# Autodesk Inventor assembly: Section 2
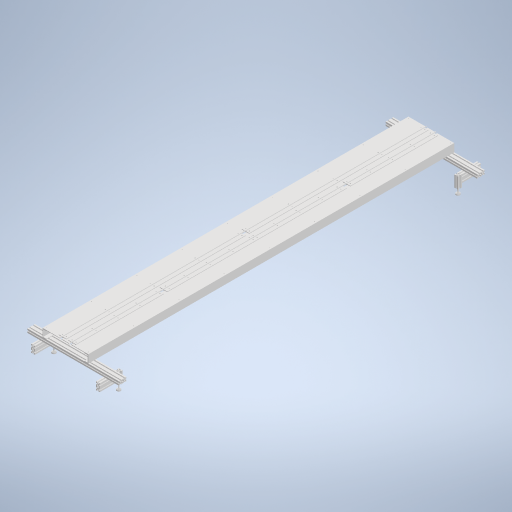
[picture p0: Inventor's stored thumbnail of the model, 512x512]
Saved by Autodesk Inventor 2023 (Build 270158030, 158C)
## iProperties
Created: 2022-06-30
Part Number: Section 2
Document SubType Name: Assembly
Designer: jeremyy
Author: jeremyy
## Documents named in this file (11)
- \\andrew.ad.cmu.edu\users\users1\jeremyy\Documents\Inventor\CMU Bridge\New folder\Section 2.iam
- \\andrew.ad.cmu.edu\users\users1\jeremyy\Documents\Inventor\CMU Bridge\New folder\VertX3in.ipt
- \\andrew.ad.cmu.edu\users\users1\jeremyy\Documents\Inventor\CMU Bridge\New folder\LongXX5.ipt
- \\andrew.ad.cmu.edu\users\users1\jeremyy\Documents\Inventor\CMU Bridge\New folder\LatXX24in.ipt
- \\andrew.ad.cmu.edu\users\users1\jeremyy\Documents\Inventor\CMU Bridge\New folder\LongC96.ipt
- \\andrew.ad.cmu.edu\users\users1\jeremyy\Documents\Inventor\CMU Bridge\New folder\Plate1ftx8ft.ipt
- \\andrew.ad.cmu.edu\users\users1\jeremyy\Documents\Inventor\CMU Bridge\New folder\Foot.ipt
- \\andrew.ad.cmu.edu\users\users1\jeremyy\Documents\Inventor\CMU Bridge\New folder\PlateRailClamp48in.iam
- \\andrew.ad.cmu.edu\users\users1\jeremyy\Documents\Inventor\CMU Bridge\New folder\PlateRail24in.iam
- \\andrew.ad.cmu.edu\users\users1\jeremyy\Documents\Inventor\CMU Bridge\New folder\RailClamp.ipt
- \\andrew.ad.cmu.edu\users\users1\jeremyy\Documents\Inventor\CMU Bridge\New folder\PlateRail23_5.iam
## Components (24 placed, 10 different names)
1. LatXX24in:1 — Flush:1, Flush:2, Mate:1, Flush:3, Mate:2, Flush:4, Mate:4, Flush:7, Flush:8, Mate:5, Flush:26
2. LongXX5:1 — Flush:1, Flush:2, Mate:1, Mate:8, Flush:15, Flush:16
3. LongXX5:2 — Flush:3, Mate:2, Flush:4, Flush:5, Flush:6, Mate:3
4. VertX3in:1 — Flush:5, Flush:6, Mate:3, Mate:13, Tangent:1
5. LongC96:1 — Mate:4, Flush:7, Flush:10, Mate:6, Flush:11
6. LongC96:2 — Flush:8, Mate:5, Flush:12, Mate:7, Flush:13, Flush:25, Flush:26
7. Plate1ftx8ft:1 — Flush:10, Mate:6, Flush:11, Flush:12, Mate:17, Flush:27, Flush:28, Mate:18, Mate:20, Flush:30, Flush:31, Mate:21, Flush:32, Flush:33, Mate:25, Mate:27
8. LatXX24in:2 — Mate:7, Flush:13, Flush:17, Flush:18, Mate:9, Mate:10, Flush:19, Flush:20, Flush:25
9. VertX3in:2 — Mate:8, Flush:15, Flush:16, Mate:14, Tangent:2
10. LongXX5:3 — Flush:17, Flush:18, Mate:9, Flush:23, Mate:12, Flush:24
11. LongXX5:4 — Mate:10, Flush:19, Flush:20, Flush:21, Mate:11, Flush:22
12. VertX3in:3 — Flush:21, Mate:11, Flush:22, Mate:16, Tangent:4
13. VertX3in:4 — Flush:23, Mate:12, Flush:24, Mate:15, Tangent:3
14. Foot:1 — Mate:13, Tangent:1
15. Foot:2 — Mate:14, Tangent:2
16. Foot:3 — Mate:15, Tangent:3
17. Foot:4 — Mate:16, Tangent:4
18. PlateRailClamp48in:1 [sub-assembly] — Mate:17, Flush:27, Flush:28, Mate:19, Flush:29
19. PlateRailClamp48in:2 [sub-assembly] — Mate:18, Mate:19, Flush:29
20. PlateRail24in:1 [sub-assembly] — Mate:20, Flush:30, Flush:31, Mate:26, Flush:34
21. PlateRail24in:2 [sub-assembly] — Mate:21, Flush:32, Flush:33, Mate:22, Mate:23, Mate:24
22. RailClamp:1 — Mate:22, Mate:23, Mate:24
23. PlateRail23_5:1 [sub-assembly] — Mate:25, Mate:26, Flush:34, Mate:28, Flush:35
24. PlateRail23_5:2 [sub-assembly] — Mate:27, Mate:28, Flush:35
## Relationships (65: Flush 33, Mate 28, Tangent 4)
- Flush:1 (-50.8 mm): LatXX24in:1 ↔ LongXX5:1
- Flush:2 (76.2 mm): LatXX24in:1 ↔ LongXX5:1
- Mate:1: LatXX24in:1 ↔ LongXX5:1
- Flush:3 (-50.8 mm): LatXX24in:1 ↔ LongXX5:2
- Mate:2: LatXX24in:1 ↔ LongXX5:2
- Flush:4 (-76.2 mm): LatXX24in:1 ↔ LongXX5:2
- Flush:5: LongXX5:2 ↔ VertX3in:1
- Flush:6: LongXX5:2 ↔ VertX3in:1
- Mate:3: LongXX5:2 ↔ VertX3in:1
- Mate:4: LatXX24in:1 ↔ LongC96:1
- Flush:7: LatXX24in:1 ↔ LongC96:1
- Flush:8: LatXX24in:1 ↔ LongC96:2
- Mate:5: LatXX24in:1 ↔ LongC96:2
- Flush:10: LongC96:1 ↔ Plate1ftx8ft:1
- Mate:6: LongC96:1 ↔ Plate1ftx8ft:1
- Flush:11: LongC96:1 ↔ Plate1ftx8ft:1
- Flush:12: LongC96:2 ↔ Plate1ftx8ft:1
- Mate:7: LongC96:2 ↔ LatXX24in:2
- Flush:13: LongC96:2 ↔ LatXX24in:2
- Mate:8: LongXX5:1 ↔ VertX3in:2
- Flush:15: LongXX5:1 ↔ VertX3in:2
- Flush:16: LongXX5:1 ↔ VertX3in:2
- Flush:17 (-50.8 mm): LatXX24in:2 ↔ LongXX5:3
- Flush:18 (76.2 mm): LatXX24in:2 ↔ LongXX5:3
- Mate:9: LatXX24in:2 ↔ LongXX5:3
- Mate:10: LatXX24in:2 ↔ LongXX5:4
- Flush:19 (76.2 mm): LatXX24in:2 ↔ LongXX5:4
- Flush:20 (-50.8 mm): LatXX24in:2 ↔ LongXX5:4
- Flush:21: LongXX5:4 ↔ VertX3in:3
- Mate:11: LongXX5:4 ↔ VertX3in:3
- Flush:22: LongXX5:4 ↔ VertX3in:3
- Flush:23: LongXX5:3 ↔ VertX3in:4
- Mate:12: LongXX5:3 ↔ VertX3in:4
- Flush:24: LongXX5:3 ↔ VertX3in:4
- Flush:25 (101.6 mm): LongC96:2 ↔ LatXX24in:2
- Flush:26 (101.6 mm): LatXX24in:1 ↔ LongC96:2
- Mate:13: VertX3in:1 ↔ Foot:1
- Tangent:1: VertX3in:1 ↔ Foot:1
- Mate:14: VertX3in:2 ↔ Foot:2
- Tangent:2: VertX3in:2 ↔ Foot:2
- Mate:15: VertX3in:4 ↔ Foot:3
- Tangent:3: VertX3in:4 ↔ Foot:3
- Mate:16: VertX3in:3 ↔ Foot:4
- Tangent:4: VertX3in:3 ↔ Foot:4
- Mate:17: Plate1ftx8ft:1 ↔ PlateRailClamp48in:1
- Flush:27: Plate1ftx8ft:1 ↔ PlateRailClamp48in:1
- Flush:28 (95.25 mm): Plate1ftx8ft:1 ↔ PlateRailClamp48in:1
- Mate:18: Plate1ftx8ft:1 ↔ PlateRailClamp48in:2
- Mate:19: PlateRailClamp48in:1 ↔ PlateRailClamp48in:2
- Flush:29: PlateRailClamp48in:1 ↔ PlateRailClamp48in:2
- Mate:20: Plate1ftx8ft:1 ↔ PlateRail24in:1
- Flush:30: Plate1ftx8ft:1 ↔ PlateRail24in:1
- Flush:31 (95.25 mm): Plate1ftx8ft:1 ↔ PlateRail24in:1
- Mate:21: Plate1ftx8ft:1 ↔ PlateRail24in:2
- Flush:32: Plate1ftx8ft:1 ↔ PlateRail24in:2
- Flush:33 (95.25 mm): Plate1ftx8ft:1 ↔ PlateRail24in:2
- Mate:22: PlateRail24in:2 ↔ RailClamp:1
- Mate:23: PlateRail24in:2 ↔ RailClamp:1
- Mate:24 (3.175 mm): PlateRail24in:2 ↔ RailClamp:1
- Mate:25: Plate1ftx8ft:1 ↔ PlateRail23_5:1
- Mate:26: PlateRail24in:1 ↔ PlateRail23_5:1
- Flush:34: PlateRail24in:1 ↔ PlateRail23_5:1
- Mate:27: Plate1ftx8ft:1 ↔ PlateRail23_5:2
- Mate:28: PlateRail23_5:1 ↔ PlateRail23_5:2
- Flush:35: PlateRail23_5:1 ↔ PlateRail23_5:2
